# Autodesk Inventor assembly: ASY MSC 900.2 support
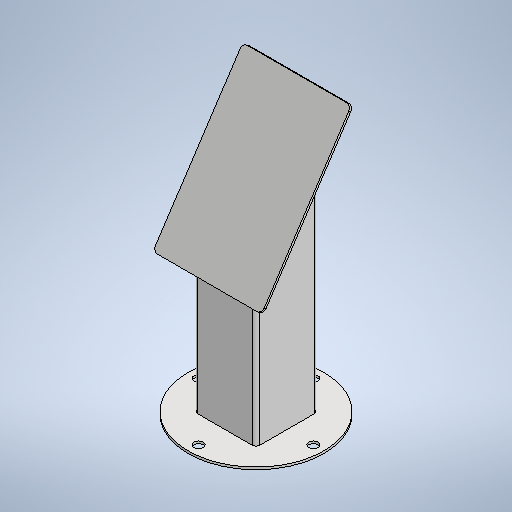
[picture p0: Inventor's stored thumbnail of the model, 512x512]
Saved by Autodesk Inventor 2025 (Build 290162010, 162A)
## iProperties
Created: 2024-08-15
Part Number: ASY MSC 900.2 support
Document SubType Name: Assembly
Designer: admin
Stock Number: ASY МОО 900.2 опора
Author: admin
Revision Number: 8
## Documents named in this file (5)
- C:\Users\admin\YandexDisk-badmisterfox\домашниий пк\Inventor\Manturovo\Manturovo_Se-clar\ASY MSC 900.2 support.iam
- C:\Users\admin\YandexDisk-badmisterfox\домашниий пк\Inventor\Manturovo\Manturovo_Se-clar\MSC 903 base tube.ipt
- C:\Users\admin\YandexDisk-badmisterfox\домашниий пк\Inventor\Manturovo\Manturovo_Se-clar\MSC 904 flange base tube.ipt
- C:\Users\admin\YandexDisk-badmisterfox\домашниий пк\Inventor\Manturovo\Manturovo_Se-clar\MSC 905 flange base tube support.ipt
- C:\Users\admin\YandexDisk-badmisterfox\домашниий пк\Inventor\Manturovo\Manturovo_Se-clar\MSC 908 tube support 3.ipt
## Components (4 placed, 4 different names)
1. MSC 903 base tube:1
2. MSC 904 flange base tube:1 — Mate:1, Mate:2, Mate:3, Mate:4
3. MSC 905 flange base tube support:1 — Rigid:3
4. MSC 908 tube support 3:1 — Rigid:3
## Relationships (7: Mate 4, WeldJoint 3)
- [WeldJoint]: MSC 903 base tube:1 ↔ MSC 904 flange base tube:1
- [WeldJoint]: MSC 903 base tube:1 ↔ MSC 905 flange base tube support:1
- Mate:1: MSC 904 flange base tube:1
- Mate:2: MSC 904 flange base tube:1
- Mate:3: MSC 904 flange base tube:1
- Mate:4: MSC 904 flange base tube:1
- Rigid:3 [WeldJoint]: MSC 905 flange base tube support:1 ↔ MSC 908 tube support 3:1
